# Autodesk Inventor assembly: Assembly Of Conveyor
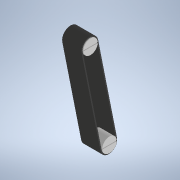
[picture p0: Inventor's stored thumbnail of the model, 180x180]
Saved by Autodesk Inventor 2022.2 (Build 262287000, 287)
## iProperties
Created: 2022-02-21
Part Number: Assembly Of Conveyor
Document SubType Name: Assembly
Designer: PRASHANTH
Author: PRASHANTH
## Documents named in this file (3)
- E:\BME\Autodesk Sample\Assembly Of Conveyor.iam
- E:\BME\Autodesk Sample\Conveyor Belt.ipt
- E:\BME\Autodesk Sample\Conveyor Driver Shaft.ipt
## Components (3 placed, 2 different names)
1. Conveyor Belt:1 — Insert:1, Insert:2
2. Conveyor Driver Shaft:1 — Insert:1, Rotation:1
3. Conveyor Driver Shaft:2 — Insert:2, Rotation:1
## Relationships (3: Insert 2, RelateRotation 1)
- Insert:1: Conveyor Belt:1 ↔ Conveyor Driver Shaft:1
- Insert:2: Conveyor Belt:1 ↔ Conveyor Driver Shaft:2
- Rotation:1 [RelateRotation] (1 ul): Conveyor Driver Shaft:1 ↔ Conveyor Driver Shaft:2
